# Autodesk Inventor assembly: 胴体_1
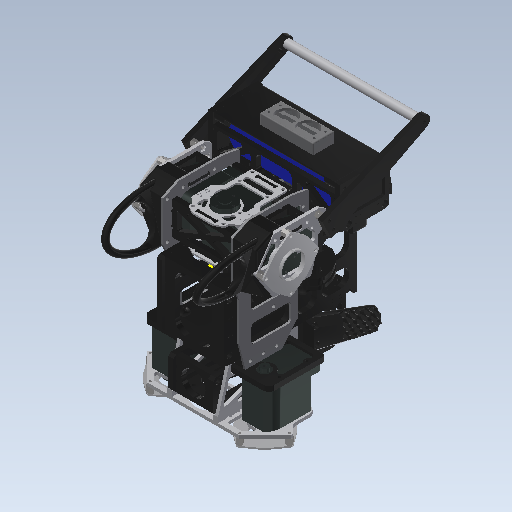
[picture p0: Inventor's stored thumbnail of the model, 512x512]
Saved by Autodesk Inventor 2020.3 (Build 243373000, 373)
## iProperties
Created: 2016-05-03
Part Number: 胴体_1
Document SubType Name: Assembly
Designer: hiroaki
Mass: 1394.39 g
Surface Area: 4542.63 cm^2
Volume: 847.153 cm^3
Density: 1.64598 g/cm^3
Author: hiroaki
## Documents named in this file (27)
- C:\Users\masato\Documents\Inventor\OpenPlatform_ver3_0\上半身\胴体\胴体_1.iam
- C:\Users\masato\Documents\Inventor\OpenPlatform_ver3_0\既製品\B3M11xx.ipt
- C:\Users\masato\Documents\Inventor\OpenPlatform_ver3_0\既製品\B3M10xx.ipt
- C:\Users\masato\Documents\Inventor\OpenPlatform_ver3_0\上半身\胴体\胴体_メインフレーム_1_1.ipt
- C:\Users\masato\Documents\Inventor\OpenPlatform_ver3_0\下半身\付け根ロール\付け根ロール_サブフレーム_1_3.ipt
- C:\Users\masato\Documents\Inventor\OpenPlatform_ver3_0\上半身\胴体\胴体_メインフレーム_1_2.ipt
- C:\Users\masato\Documents\Inventor\OpenPlatform_ver3_0\上半身\胴体\胴体_サブフレーム_1_1.ipt
- C:\Users\masato\Documents\Inventor\OpenPlatform_ver3_0\上半身\胴体\胴体_サブフレーム_1_2.ipt
- C:\Users\masato\Documents\Inventor\OpenPlatform_ver3_0\上半身\胴体\胴体_サブフレーム_1_3.ipt
- C:\Users\masato\Documents\Inventor\OpenPlatform_ver3_0\上半身\胴体\胴体_サブフレーム_1_4.ipt
- C:\Users\masato\Documents\Inventor\OpenPlatform_ver3_0\上半身\胴体\胴体_サブフレーム_1_1_MIR.ipt
- C:\Users\masato\Documents\Inventor\OpenPlatform_ver3_0\上半身\胴体\胴体_サブフレーム_1_9.ipt
- C:\Users\masato\Documents\Inventor\OpenPlatform_ver3_0\上半身\胴体\胴体_メインフレーム_1_12.ipt
- C:\Users\masato\Documents\Inventor\OpenPlatform_ver3_0\上半身\胴体\胴体_メインフレーム_1_13.ipt
- C:\Users\masato\Documents\Inventor\OpenPlatform_ver3_0\上半身\胴体\胴体_サブフレーム_1_10.ipt
- C:\Users\masato\Documents\Inventor\OpenPlatform_ver3_0\上半身\胴体\胴体_サブフレーム_1_11.ipt
- C:\Users\masato\Documents\Inventor\OpenPlatform_ver3_0\既製品\SLCG5_5-6.ipt
- C:\Users\masato\Documents\Inventor\OpenPlatform_ver3_0\既製品\ALSFB6-66.ipt
- C:\Users\masato\Documents\Inventor\OpenPlatform_ver3_0\上半身\コックピット\コックピット_2\コックピット_2.iam
- C:\Users\masato\Documents\Inventor\OpenPlatform_ver3_0\上半身\胴体\胴体_サブフレーム_1_12.ipt
- C:\Users\masato\Documents\Inventor\OpenPlatform_ver3_0\既製品\AETTF8-135-M3-N3.ipt
- C:\Users\masato\Documents\Inventor\OpenPlatform_ver3_0\既製品\SLCG5_5-8.ipt
- C:\Users\masato\Documents\Inventor\OpenPlatform_ver3_0\上半身\胴体\胴体_サブフレーム_1_4_MIR.ipt
- C:\Users\masato\Documents\Inventor\OpenPlatform_ver3_0\上半身\胴体\RearBumper_Lower.ipt
- C:\Users\masato\Documents\Inventor\OpenPlatform_ver3_0\上半身\胴体\RearBumper_Lower_MIR.ipt
- C:\Users\masato\Documents\Inventor\OpenPlatform_ver3_0\上半身\胴体\FrontBumper_MIR.iam
- C:\Users\masato\Documents\Inventor\OpenPlatform_ver3_0\上半身\胴体\FrontBumper.iam
## Components (60 placed, 25 different names)
1. 胴体_メインフレーム_1_1:1 — 挿入:1, 挿入:2, 挿入:3, 挿入:4, 挿入:5, 挿入:6, 挿入:43, 挿入:44, 挿入:120, 挿入:121, 挿入:194, 挿入:195, 挿入:196, 挿入:197, 挿入:198, 挿入:199, 挿入:200, 挿入:201
2. 付け根ロール_サブフレーム_1_3:1 — 挿入:218, 挿入:219, 挿入:220, 挿入:221
3. 胴体_メインフレーム_1_2:1 — 挿入:23, 挿入:24, 挿入:25, 挿入:28
4. 胴体_メインフレーム_1_12:1 — 挿入:148, 挿入:149, 挿入:150, 挿入:151, メイト:13, メイト:16
5. 胴体_サブフレーム_1_1:1 — 挿入:43, 挿入:44, メイト:9, メイト:10, メイト:11, 角度:49, 挿入:275, 挿入:276
6. 胴体_サブフレーム_1_2:1 — フラッシュ:1, メイト:3, メイト:4
7. 胴体_サブフレーム_1_3:1 — 挿入:150, 挿入:151, 挿入:162, 挿入:163, 挿入:168, 挿入:169, 挿入:192, 挿入:193, 挿入:228, 挿入:229, メイト:4, 挿入:236, 挿入:254, メイト:12
8. 胴体_サブフレーム_1_4:1 — 挿入:57, 挿入:58, 挿入:148, 挿入:149, 挿入:152, 挿入:153, 挿入:206, 挿入:207, 挿入:208, 挿入:209, 挿入:248, 挿入:249, 角度:47, 角度:48
9. 胴体_サブフレーム_1_9:1 — 挿入:133, 挿入:134, 挿入:135
10. 胴体_サブフレーム_1_10:1 — 挿入:173, 挿入:174, 挿入:175, 挿入:176, 挿入:179, 挿入:188, 挿入:189
11. 胴体_サブフレーム_1_11:1 — 挿入:182, 挿入:183, 挿入:184, 挿入:185, 挿入:186, 挿入:187
12. 胴体_サブフレーム_1_12:1 — 挿入:247, 挿入:250, 挿入:251
13. 胴体_メインフレーム_1_13:1 — 挿入:188, 挿入:189, 挿入:190, 挿入:191, 挿入:192, 挿入:193
14. B3M11xx:5 — 挿入:175, 挿入:176, 挿入:179, 挿入:182, 挿入:183, 挿入:185, 挿入:186
15. B3M11xx:4 — 挿入:57, 挿入:58, 挿入:133, 挿入:134, 挿入:135, 角度:31, 角度:39
16. B3M11xx:3 — 角度:1, 挿入:130, 挿入:131, 挿入:132, 挿入:264, 挿入:265, 挿入:266
17. B3M11xx:2 — 挿入:2, 挿入:4, 挿入:5, 挿入:23, 挿入:25, 角度:23, 角度:43
18. B3M11xx:1 — 角度:1, 挿入:1, 挿入:3, 挿入:6, 挿入:24, 挿入:28
19. SLCG5_5-6:1 — 挿入:200, 挿入:218, 角度:27, 角度:29
20. SLCG5_5-6:2 — 挿入:196, 挿入:222, 角度:25, 角度:28, 角度:43
21. SLCG5_5-6:3 — 挿入:198, 挿入:220, 角度:29
22. SLCG5_5-6:4 — 挿入:199, 挿入:219, 角度:30
23. SLCG5_5-6:5 — 挿入:217, 角度:34, 挿入:272
24. SLCG5_5-6:6 — 挿入:216, 角度:42, 挿入:271
25. SLCG5_5-6:7 — 挿入:197, 挿入:225, 角度:26
26. SLCG5_5-6:8 — 挿入:201, 挿入:221, 角度:28, 角度:30
27. SLCG5_5-6:9 — 挿入:206, 挿入:212, 角度:40
28. SLCG5_5-6:10 — 挿入:215, 角度:41, 挿入:269
29. SLCG5_5-6:11 — 挿入:214, 角度:33, 角度:34, 挿入:270
30. SLCG5_5-6:12 — 挿入:195, 挿入:224, 角度:25
31. SLCG5_5-6:13 — 挿入:207, 挿入:213, 角度:32
32. SLCG5_5-6:14 — 挿入:208, 挿入:211, 角度:31, 角度:32, 角度:33
33. SLCG5_5-6:15 — 挿入:209, 挿入:210, 角度:39, 角度:40, 角度:41, 角度:42
34. SLCG5_5-6:16 — 挿入:194, 挿入:223, 角度:23, 角度:26, 角度:27
35. ALSFB6-66:1 — 挿入:229, 挿入:230, メイト:3, メイト:9
36. ALSFB6-66:2 — 挿入:227, 挿入:228, メイト:1, メイト:2
37. ALSFB6-66:3 — メイト:10, メイト:11, 挿入:235, 挿入:236
38. コックピット_2:1 [sub-assembly] — 挿入:254, 挿入:255, 角度:49
39. AETTF8-135-M3-N3:1 — 挿入:246, 挿入:247
40. SLCG5_5-8:1 — 挿入:252, 挿入:262
41. SLCG5_5-8:2 — 挿入:249, 挿入:251, 角度:48
42. SLCG5_5-8:3 — 挿入:253, 挿入:263
43. SLCG5_5-8:4 — 挿入:248, 挿入:250, 角度:47
44. 胴体_サブフレーム_1_12:2 — 挿入:246, 挿入:252, 挿入:253
45. 胴体_メインフレーム_1_13:2 — 挿入:168, 挿入:169, 挿入:170, 挿入:171, 挿入:173, 挿入:174, 挿入:184, 挿入:187
46. 胴体_メインフレーム_1_12:2 — 挿入:152, 挿入:153, 挿入:162, 挿入:163
47. 胴体_メインフレーム_1_12:3 — 挿入:156, 挿入:157, 挿入:267, 挿入:268
48. 胴体_メインフレーム_1_12:4 — 挿入:160, 挿入:161, 挿入:260, 挿入:261, メイト:15, メイト:17
49. 胴体_サブフレーム_1_9:2 — 挿入:130, 挿入:131, 挿入:132
50. 付け根ロール_サブフレーム_1_3:2 — 挿入:222, 挿入:223, 挿入:224, 挿入:225
51. 付け根ロール_サブフレーム_1_3:3 — 挿入:210, 挿入:211, 挿入:212, 挿入:213
52. 付け根ロール_サブフレーム_1_3:4 — 挿入:214, 挿入:215, 挿入:216, 挿入:217
53. 胴体_サブフレーム_1_1_MIR:1 — 挿入:120, 挿入:121, メイト:7, 挿入:273, 挿入:274
54. 胴体_サブフレーム_1_2:2 — メイト:1, フラッシュ:1, メイト:2, メイト:5, メイト:7
55. 胴体_サブフレーム_1_3:2 — 挿入:156, 挿入:157, 挿入:160, 挿入:161, 挿入:170, 挿入:171, 挿入:190, 挿入:191, 挿入:227, 挿入:230, メイト:5, 挿入:235, 挿入:255, メイト:14
56. 胴体_サブフレーム_1_4_MIR:1 — 挿入:260, 挿入:261, 挿入:262, 挿入:263, 挿入:264, 挿入:265, 挿入:266, 挿入:267, 挿入:268, 挿入:269, 挿入:270, 挿入:271, 挿入:272
57. RearBumper_Lower:1 — 挿入:275, 挿入:276
58. RearBumper_Lower_MIR:1 — 挿入:273, 挿入:274
59. FrontBumper_MIR:1 [sub-assembly] — メイト:12, メイト:13, メイト:16
60. FrontBumper:1 [sub-assembly] — メイト:14, メイト:15, メイト:17
## Relationships (152: Insert 116, Angle 20, Mate 15, Flush 1)
- 角度:1 [Angle] (0 deg): B3M11xx:3 ↔ B3M11xx:1
- 挿入:1 [Insert]: 胴体_メインフレーム_1_1:1 ↔ B3M11xx:1
- 挿入:2 [Insert]: 胴体_メインフレーム_1_1:1 ↔ B3M11xx:2
- 挿入:3 [Insert]: 胴体_メインフレーム_1_1:1 ↔ B3M11xx:1
- 挿入:4 [Insert]: 胴体_メインフレーム_1_1:1 ↔ B3M11xx:2
- 挿入:5 [Insert]: 胴体_メインフレーム_1_1:1 ↔ B3M11xx:2
- 挿入:6 [Insert]: 胴体_メインフレーム_1_1:1 ↔ B3M11xx:1
- 挿入:23 [Insert]: 胴体_メインフレーム_1_2:1 ↔ B3M11xx:2
- 挿入:24 [Insert]: 胴体_メインフレーム_1_2:1 ↔ B3M11xx:1
- 挿入:25 [Insert]: 胴体_メインフレーム_1_2:1 ↔ B3M11xx:2
- 挿入:28 [Insert]: 胴体_メインフレーム_1_2:1 ↔ B3M11xx:1
- 挿入:43 [Insert]: 胴体_メインフレーム_1_1:1 ↔ 胴体_サブフレーム_1_1:1
- 挿入:44 [Insert]: 胴体_メインフレーム_1_1:1 ↔ 胴体_サブフレーム_1_1:1
- 挿入:57 [Insert]: 胴体_サブフレーム_1_4:1 ↔ B3M11xx:4
- 挿入:58 [Insert]: 胴体_サブフレーム_1_4:1 ↔ B3M11xx:4
- 挿入:120 [Insert]: 胴体_メインフレーム_1_1:1 ↔ 胴体_サブフレーム_1_1_MIR:1
- 挿入:121 [Insert]: 胴体_メインフレーム_1_1:1 ↔ 胴体_サブフレーム_1_1_MIR:1
- 挿入:130 [Insert]: B3M11xx:3 ↔ 胴体_サブフレーム_1_9:2
- 挿入:131 [Insert]: B3M11xx:3 ↔ 胴体_サブフレーム_1_9:2
- 挿入:132 [Insert]: B3M11xx:3 ↔ 胴体_サブフレーム_1_9:2
- 挿入:133 [Insert]: 胴体_サブフレーム_1_9:1 ↔ B3M11xx:4
- 挿入:134 [Insert]: 胴体_サブフレーム_1_9:1 ↔ B3M11xx:4
- 挿入:135 [Insert]: 胴体_サブフレーム_1_9:1 ↔ B3M11xx:4
- 挿入:148 [Insert]: 胴体_メインフレーム_1_12:1 ↔ 胴体_サブフレーム_1_4:1
- 挿入:149 [Insert]: 胴体_メインフレーム_1_12:1 ↔ 胴体_サブフレーム_1_4:1
- 挿入:150 [Insert]: 胴体_メインフレーム_1_12:1 ↔ 胴体_サブフレーム_1_3:1
- 挿入:151 [Insert]: 胴体_メインフレーム_1_12:1 ↔ 胴体_サブフレーム_1_3:1
- 挿入:152 [Insert]: 胴体_サブフレーム_1_4:1 ↔ 胴体_メインフレーム_1_12:2
- 挿入:153 [Insert]: 胴体_サブフレーム_1_4:1 ↔ 胴体_メインフレーム_1_12:2
- 挿入:156 [Insert]: 胴体_メインフレーム_1_12:3 ↔ 胴体_サブフレーム_1_3:2
- 挿入:157 [Insert]: 胴体_メインフレーム_1_12:3 ↔ 胴体_サブフレーム_1_3:2
- 挿入:160 [Insert]: 胴体_メインフレーム_1_12:4 ↔ 胴体_サブフレーム_1_3:2
- 挿入:161 [Insert]: 胴体_メインフレーム_1_12:4 ↔ 胴体_サブフレーム_1_3:2
- 挿入:162 [Insert]: 胴体_サブフレーム_1_3:1 ↔ 胴体_メインフレーム_1_12:2
- 挿入:163 [Insert]: 胴体_サブフレーム_1_3:1 ↔ 胴体_メインフレーム_1_12:2
- 挿入:168 [Insert]: 胴体_サブフレーム_1_3:1 ↔ 胴体_メインフレーム_1_13:2
- 挿入:169 [Insert]: 胴体_サブフレーム_1_3:1 ↔ 胴体_メインフレーム_1_13:2
- 挿入:170 [Insert]: 胴体_メインフレーム_1_13:2 ↔ 胴体_サブフレーム_1_3:2
- 挿入:171 [Insert]: 胴体_メインフレーム_1_13:2 ↔ 胴体_サブフレーム_1_3:2
- 挿入:173 [Insert]: 胴体_サブフレーム_1_10:1 ↔ 胴体_メインフレーム_1_13:2
- 挿入:174 [Insert]: 胴体_サブフレーム_1_10:1 ↔ 胴体_メインフレーム_1_13:2
- 挿入:175 [Insert]: 胴体_サブフレーム_1_10:1 ↔ B3M11xx:5
- 挿入:176 [Insert]: 胴体_サブフレーム_1_10:1 ↔ B3M11xx:5
- 挿入:179 [Insert]: 胴体_サブフレーム_1_10:1 ↔ B3M11xx:5
- 挿入:182 [Insert]: 胴体_サブフレーム_1_11:1 ↔ B3M11xx:5
- 挿入:183 [Insert]: 胴体_サブフレーム_1_11:1 ↔ B3M11xx:5
- 挿入:184 [Insert]: 胴体_サブフレーム_1_11:1 ↔ 胴体_メインフレーム_1_13:2
- 挿入:185 [Insert]: 胴体_サブフレーム_1_11:1 ↔ B3M11xx:5
- 挿入:186 [Insert]: 胴体_サブフレーム_1_11:1 ↔ B3M11xx:5
- 挿入:187 [Insert]: 胴体_サブフレーム_1_11:1 ↔ 胴体_メインフレーム_1_13:2
- 挿入:188 [Insert]: 胴体_サブフレーム_1_10:1 ↔ 胴体_メインフレーム_1_13:1
- 挿入:189 [Insert]: 胴体_サブフレーム_1_10:1 ↔ 胴体_メインフレーム_1_13:1
- 挿入:190 [Insert]: 胴体_メインフレーム_1_13:1 ↔ 胴体_サブフレーム_1_3:2
- 挿入:191 [Insert]: 胴体_メインフレーム_1_13:1 ↔ 胴体_サブフレーム_1_3:2
- 挿入:192 [Insert]: 胴体_サブフレーム_1_3:1 ↔ 胴体_メインフレーム_1_13:1
- 挿入:193 [Insert]: 胴体_サブフレーム_1_3:1 ↔ 胴体_メインフレーム_1_13:1
- 挿入:194 [Insert]: 胴体_メインフレーム_1_1:1 ↔ SLCG5_5-6:16
- 挿入:195 [Insert]: 胴体_メインフレーム_1_1:1 ↔ SLCG5_5-6:12
- 挿入:196 [Insert]: 胴体_メインフレーム_1_1:1 ↔ SLCG5_5-6:2
- 挿入:197 [Insert]: 胴体_メインフレーム_1_1:1 ↔ SLCG5_5-6:7
- 挿入:198 [Insert]: 胴体_メインフレーム_1_1:1 ↔ SLCG5_5-6:3
- 挿入:199 [Insert]: 胴体_メインフレーム_1_1:1 ↔ SLCG5_5-6:4
- 挿入:200 [Insert]: 胴体_メインフレーム_1_1:1 ↔ SLCG5_5-6:1
- 挿入:201 [Insert]: 胴体_メインフレーム_1_1:1 ↔ SLCG5_5-6:8
- 挿入:206 [Insert]: 胴体_サブフレーム_1_4:1 ↔ SLCG5_5-6:9
- 挿入:207 [Insert]: 胴体_サブフレーム_1_4:1 ↔ SLCG5_5-6:13
- 挿入:208 [Insert]: 胴体_サブフレーム_1_4:1 ↔ SLCG5_5-6:14
- 挿入:209 [Insert]: 胴体_サブフレーム_1_4:1 ↔ SLCG5_5-6:15
- 挿入:210 [Insert]: SLCG5_5-6:15 ↔ 付け根ロール_サブフレーム_1_3:3
- 挿入:211 [Insert]: SLCG5_5-6:14 ↔ 付け根ロール_サブフレーム_1_3:3
- 挿入:212 [Insert]: SLCG5_5-6:9 ↔ 付け根ロール_サブフレーム_1_3:3
- 挿入:213 [Insert]: SLCG5_5-6:13 ↔ 付け根ロール_サブフレーム_1_3:3
- 挿入:214 [Insert]: SLCG5_5-6:11 ↔ 付け根ロール_サブフレーム_1_3:4
- 挿入:215 [Insert]: SLCG5_5-6:10 ↔ 付け根ロール_サブフレーム_1_3:4
- 挿入:216 [Insert]: SLCG5_5-6:6 ↔ 付け根ロール_サブフレーム_1_3:4
- 挿入:217 [Insert]: SLCG5_5-6:5 ↔ 付け根ロール_サブフレーム_1_3:4
- 挿入:218 [Insert]: 付け根ロール_サブフレーム_1_3:1 ↔ SLCG5_5-6:1
- 挿入:219 [Insert]: 付け根ロール_サブフレーム_1_3:1 ↔ SLCG5_5-6:4
- 挿入:220 [Insert]: 付け根ロール_サブフレーム_1_3:1 ↔ SLCG5_5-6:3
- 挿入:221 [Insert]: 付け根ロール_サブフレーム_1_3:1 ↔ SLCG5_5-6:8
- 挿入:222 [Insert]: SLCG5_5-6:2 ↔ 付け根ロール_サブフレーム_1_3:2
- 挿入:223 [Insert]: SLCG5_5-6:16 ↔ 付け根ロール_サブフレーム_1_3:2
- 挿入:224 [Insert]: SLCG5_5-6:12 ↔ 付け根ロール_サブフレーム_1_3:2
- 挿入:225 [Insert]: SLCG5_5-6:7 ↔ 付け根ロール_サブフレーム_1_3:2
- 角度:23 [Angle] (0 deg): B3M11xx:2 ↔ SLCG5_5-6:16
- 角度:25 [Angle] (0 deg): SLCG5_5-6:2 ↔ SLCG5_5-6:12
- 角度:26 [Angle] (0 deg): SLCG5_5-6:7 ↔ SLCG5_5-6:16
- 角度:27 [Angle] (0 deg): SLCG5_5-6:1 ↔ SLCG5_5-6:16
- 角度:28 [Angle] (0 deg): SLCG5_5-6:2 ↔ SLCG5_5-6:8
- 角度:29 [Angle] (0 deg): SLCG5_5-6:1 ↔ SLCG5_5-6:3
- 角度:30 [Angle] (0 deg): SLCG5_5-6:4 ↔ SLCG5_5-6:8
- 角度:31 [Angle] (0 deg): B3M11xx:4 ↔ SLCG5_5-6:14
- 角度:32 [Angle] (0 deg): SLCG5_5-6:13 ↔ SLCG5_5-6:14
- 角度:33 [Angle] (0 deg): SLCG5_5-6:11 ↔ SLCG5_5-6:14
- 角度:34 [Angle] (0 deg): SLCG5_5-6:5 ↔ SLCG5_5-6:11
- 挿入:227 [Insert]: ALSFB6-66:2 ↔ 胴体_サブフレーム_1_3:2
- 挿入:228 [Insert]: 胴体_サブフレーム_1_3:1 ↔ ALSFB6-66:2
- 挿入:229 [Insert]: 胴体_サブフレーム_1_3:1 ↔ ALSFB6-66:1
- 挿入:230 [Insert]: ALSFB6-66:1 ↔ 胴体_サブフレーム_1_3:2
- メイト:1 [Mate] (0.005 mm): ALSFB6-66:2 ↔ 胴体_サブフレーム_1_2:2
- フラッシュ:1 [Flush]: 胴体_サブフレーム_1_2:1 ↔ 胴体_サブフレーム_1_2:2
- メイト:2 [Mate] (0.05 mm): ALSFB6-66:2 ↔ 胴体_サブフレーム_1_2:2
- メイト:3 [Mate] (0.005 mm): 胴体_サブフレーム_1_2:1 ↔ ALSFB6-66:1
- メイト:4 [Mate]: 胴体_サブフレーム_1_2:1 ↔ 胴体_サブフレーム_1_3:1
- メイト:5 [Mate]: 胴体_サブフレーム_1_2:2 ↔ 胴体_サブフレーム_1_3:2
- メイト:7 [Mate]: 胴体_サブフレーム_1_1_MIR:1 ↔ 胴体_サブフレーム_1_2:2
- メイト:9 [Mate] (0.005 mm): 胴体_サブフレーム_1_1:1 ↔ ALSFB6-66:1
- メイト:10 [Mate] (0.005 mm): 胴体_サブフレーム_1_1:1 ↔ ALSFB6-66:3
- メイト:11 [Mate] (0.005 mm): 胴体_サブフレーム_1_1:1 ↔ ALSFB6-66:3
- 挿入:235 [Insert]: ALSFB6-66:3 ↔ 胴体_サブフレーム_1_3:2
- 挿入:236 [Insert]: 胴体_サブフレーム_1_3:1 ↔ ALSFB6-66:3
- 挿入:246 [Insert]: AETTF8-135-M3-N3:1 ↔ 胴体_サブフレーム_1_12:2
- 挿入:247 [Insert]: 胴体_サブフレーム_1_12:1 ↔ AETTF8-135-M3-N3:1
- 挿入:248 [Insert]: 胴体_サブフレーム_1_4:1 ↔ SLCG5_5-8:4
- 挿入:249 [Insert]: 胴体_サブフレーム_1_4:1 ↔ SLCG5_5-8:2
- 挿入:250 [Insert]: 胴体_サブフレーム_1_12:1 ↔ SLCG5_5-8:4
- 挿入:251 [Insert]: 胴体_サブフレーム_1_12:1 ↔ SLCG5_5-8:2
- 挿入:252 [Insert]: SLCG5_5-8:1 ↔ 胴体_サブフレーム_1_12:2
- 挿入:253 [Insert]: SLCG5_5-8:3 ↔ 胴体_サブフレーム_1_12:2
- 角度:39 [Angle] (0 deg): B3M11xx:4 ↔ SLCG5_5-6:15
- 角度:40 [Angle] (0 deg): SLCG5_5-6:9 ↔ SLCG5_5-6:15
- 角度:41 [Angle] (0 deg): SLCG5_5-6:10 ↔ SLCG5_5-6:15
- 角度:42 [Angle] (0 deg): SLCG5_5-6:6 ↔ SLCG5_5-6:15
- 角度:43 [Angle] (0 deg): B3M11xx:2 ↔ SLCG5_5-6:2
- 角度:47 [Angle] (0 deg): 胴体_サブフレーム_1_4:1 ↔ SLCG5_5-8:4
- 角度:48 [Angle] (0 deg): 胴体_サブフレーム_1_4:1 ↔ SLCG5_5-8:2
- 挿入:254 [Insert]: 胴体_サブフレーム_1_3:1 ↔ コックピット_2:1
- 挿入:255 [Insert]: コックピット_2:1 ↔ 胴体_サブフレーム_1_3:2
- 角度:49 [Angle] (180 deg): 胴体_サブフレーム_1_1:1 ↔ コックピット_2:1
- 挿入:260 [Insert]: 胴体_メインフレーム_1_12:4 ↔ 胴体_サブフレーム_1_4_MIR:1
- 挿入:261 [Insert]: 胴体_メインフレーム_1_12:4 ↔ 胴体_サブフレーム_1_4_MIR:1
- 挿入:262 [Insert]: SLCG5_5-8:1 ↔ 胴体_サブフレーム_1_4_MIR:1
- 挿入:263 [Insert]: SLCG5_5-8:3 ↔ 胴体_サブフレーム_1_4_MIR:1
- 挿入:264 [Insert]: B3M11xx:3 ↔ 胴体_サブフレーム_1_4_MIR:1
- 挿入:265 [Insert]: B3M11xx:3 ↔ 胴体_サブフレーム_1_4_MIR:1
- 挿入:266 [Insert]: B3M11xx:3 ↔ 胴体_サブフレーム_1_4_MIR:1
- 挿入:267 [Insert]: 胴体_メインフレーム_1_12:3 ↔ 胴体_サブフレーム_1_4_MIR:1
- 挿入:268 [Insert]: 胴体_メインフレーム_1_12:3 ↔ 胴体_サブフレーム_1_4_MIR:1
- 挿入:269 [Insert]: SLCG5_5-6:10 ↔ 胴体_サブフレーム_1_4_MIR:1
- 挿入:270 [Insert]: SLCG5_5-6:11 ↔ 胴体_サブフレーム_1_4_MIR:1
- 挿入:271 [Insert]: SLCG5_5-6:6 ↔ 胴体_サブフレーム_1_4_MIR:1
- 挿入:272 [Insert]: SLCG5_5-6:5 ↔ 胴体_サブフレーム_1_4_MIR:1
- メイト:12 [Mate]: 胴体_サブフレーム_1_3:1 ↔ FrontBumper_MIR:1
- メイト:13 [Mate]: 胴体_メインフレーム_1_12:1 ↔ FrontBumper_MIR:1
- メイト:14 [Mate]: 胴体_サブフレーム_1_3:2 ↔ FrontBumper:1
- メイト:15 [Mate]: 胴体_メインフレーム_1_12:4 ↔ FrontBumper:1
- 挿入:273 [Insert]: 胴体_サブフレーム_1_1_MIR:1 ↔ RearBumper_Lower_MIR:1
- 挿入:274 [Insert]: 胴体_サブフレーム_1_1_MIR:1 ↔ RearBumper_Lower_MIR:1
- 挿入:275 [Insert]: 胴体_サブフレーム_1_1:1 ↔ RearBumper_Lower:1
- 挿入:276 [Insert]: 胴体_サブフレーム_1_1:1 ↔ RearBumper_Lower:1
- メイト:16 [Mate]: 胴体_メインフレーム_1_12:1 ↔ FrontBumper_MIR:1
- メイト:17 [Mate]: 胴体_メインフレーム_1_12:4 ↔ FrontBumper:1
